# Autodesk Inventor assembly: CableHolder_ASM
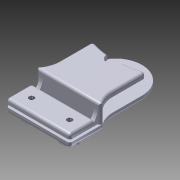
[picture p0: Inventor's stored thumbnail of the model, 180x180]
Saved by Autodesk Inventor 2014 SP1 (Build 180222100, 222)
## iProperties
Created: 2013-11-09
Part Number: CableHolder_ASM
Document SubType Name: Assembly
Designer: JustinIndra
Author: JustinIndra
## Documents named in this file (3)
- C:\Users\JustinIndra\Dropbox\Projects\Mechatronics\Camera Slider\MotorizeKamerar\MECHANICAL\CableHolder_ASM.iam
- C:\Users\JustinIndra\Dropbox\Projects\Mechatronics\Camera Slider\MotorizeKamerar\MECHANICAL\CableHolder.ipt
- C:\Users\JustinIndra\Dropbox\Projects\Mechatronics\Camera Slider\MotorizeKamerar\MECHANICAL\CableHolder02.ipt
## Components (2 placed, 2 different names)
1. CableHolder:1 — Mate:1, Mate:2, Mate:3
2. CableHolder02:1 — Mate:1, Mate:2, Mate:3
## Relationships (3: Mate 3)
- Mate:1: CableHolder:1 ↔ CableHolder02:1
- Mate:2: CableHolder:1 ↔ CableHolder02:1
- Mate:3 (1 mm): CableHolder:1 ↔ CableHolder02:1
